# Autodesk Inventor assembly: !structure
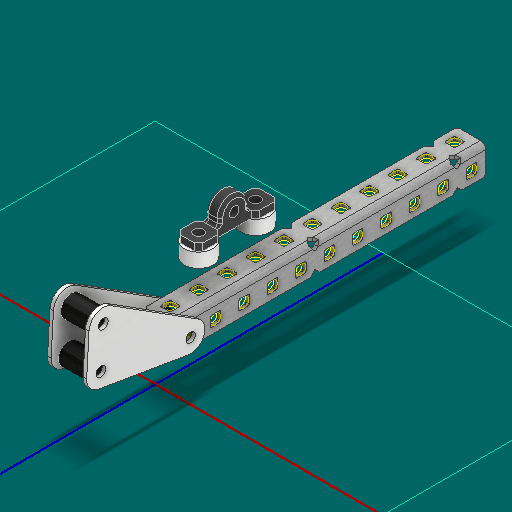
[picture p0: Inventor's stored thumbnail of the model, 512x512]
Saved by Autodesk Inventor 2025 (Build 290162000, 162)
## iProperties
Created: 2024-08-19
Part Number: !structure
Document SubType Name: Assembly
Designer: averey
Author: averey
## Documents named in this file (10)
- C:\Users\avere\vex_robotics_high_stakes\hardware\cad\ATLAS\intake\second_stage\structure\!structure.iam
- C:\Users\avere\vex_robotics_high_stakes\hardware\cad\ATLAS\intake\second_stage\structure\custom_parts\gusset.ipt
- C:\Users\avere\vex_robotics_high_stakes\hardware\cad\VEX-CAD-Inventor\Structure\Angle\Aluminum 1x1\Alu Angle 1x1x11.ipt
- C:\Users\avere\vex_robotics_high_stakes\hardware\cad\VEX-CAD-Inventor\Motion\Spacers\Spacer Nylon .375 OD\NSpacer .375 OD x .500.ipt
- C:\Users\avere\vex_robotics_high_stakes\hardware\cad\VEX-CAD-Inventor\Motion\Spacers\Spacer Nylon .375 OD.ipt
- C:\Users\avere\vex_robotics_high_stakes\hardware\cad\VEX-CAD-Inventor\Motion\Spacers\Washer Steel\SWasher .375 OD x .062500.ipt
- C:\Users\avere\vex_robotics_high_stakes\hardware\cad\VEX-CAD-Inventor\Motion\Spacers\Washer Steel.ipt
- C:\Users\avere\vex_robotics_high_stakes\hardware\cad\VEX-CAD-Inventor\Motion\Shaft LS\LS Pillow Bearing Block.ipt
- C:\Users\avere\vex_robotics_high_stakes\hardware\cad\VEX-CAD-Inventor\Motion\Spacers\Spacer Nylon .500 OD\NSpacer White .500 OD x .250.ipt
- C:\Users\avere\vex_robotics_high_stakes\hardware\cad\VEX-CAD-Inventor\Motion\Spacers\Spacer Nylon .500 OD.ipt
## Components (10 placed, 6 different names)
1. gusset:1 — Insert:4, Insert:6, Insert:17
2. gusset:2 — Angle:1, Mate:2, Insert:13
3. Alu Angle 1x1x11:1 — Angle:1, Angle:2, Insert:17, Insert:18, Mate:3
4. NSpacer .375 OD x .500:1 — Insert:4
5. NSpacer .375 OD x .500:3 — Insert:6
6. SWasher .375 OD x .062500:2 — Insert:12
7. NSpacer .375 OD x .500:4 — Insert:12, Insert:13
8. LS Pillow Bearing Block:1 — Insert:19, Insert:20
9. NSpacer White .500 OD x .250:1 — Insert:18, Insert:19
10. NSpacer White .500 OD x .250:2 — Insert:20, Mate:3
## Relationships (14: Insert 9, Mate 3, Angle 2)
- [Insert] (14.2875 mm): gusset:1 ↔ gusset:2
- [Mate]: gusset:1 ↔ gusset:2
- Angle:1 (9.6283 deg): gusset:2 ↔ Alu Angle 1x1x11:1
- Mate:2: gusset:2
- Angle:2 (0 deg): Alu Angle 1x1x11:1
- Insert:4: gusset:1 ↔ NSpacer .375 OD x .500:1
- Insert:6: gusset:1 ↔ NSpacer .375 OD x .500:3
- Insert:12: SWasher .375 OD x .062500:2 ↔ NSpacer .375 OD x .500:4
- Insert:13: gusset:2 ↔ NSpacer .375 OD x .500:4
- Insert:17: gusset:1 ↔ Alu Angle 1x1x11:1
- Insert:18 (12.7 mm): Alu Angle 1x1x11:1 ↔ NSpacer White .500 OD x .250:1
- Insert:19: LS Pillow Bearing Block:1 ↔ NSpacer White .500 OD x .250:1
- Insert:20: LS Pillow Bearing Block:1 ↔ NSpacer White .500 OD x .250:2
- Mate:3: Alu Angle 1x1x11:1 ↔ NSpacer White .500 OD x .250:2
